# Autodesk Inventor assembly: Final2
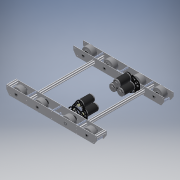
[picture p0: Inventor's stored thumbnail of the model, 180x180]
Saved by Autodesk Inventor 2016 (Build 200138000, 138)
## iProperties
Created: 2017-01-21
Part Number: Final2
Document SubType Name: Assembly
Designer: hamblettk
Author: hamblettk
## Documents named in this file (9)
- E:\1073CAD\Robot2017\DriveTrain\Final2.iam
- E:\1073CAD\Robot2017\DriveTrain\OutsidePlate2.ipt
- E:\1073CAD\Robot2017\DriveTrain\Individual Parts\3.625Churro.ipt
- E:\1073CAD\Robot2017\DriveTrain\Individual Parts\Mock 8020 3.375in.ipt
- E:\1073CAD\Robot2017\DriveTrain\InsidePlate2.ipt
- E:\1073CAD\Robot2017\DriveTrain\Individual Parts\Mock 8020 28.25in.ipt
- E:\1073CAD\Robot2017\DriveTrain\Individual Parts\DoublePulleyGearbox.iam
- E:\1073CAD\Robot2017\DriveTrain\Individual Parts\SinglePulley.iam
- E:\1073CAD\Robot2017\DriveTrain\Individual Parts\DoublePulley.iam
## Components (32 placed, 8 different names)
1. OutsidePlate2:1 — Mate:1, Mate:2, Mate:3, Mate:4, Mate:5, Mate:6, Mate:7, Mate:8, Mate:9, Mate:10, Flush:1, Flush:2, Mate:12, Mate:13, Mate:29, Mate:30, Mate:32, Mate:33, Mate:36, Mate:37, Mate:40, Mate:41
2. 3.625Churro:1 — Mate:1
3. 3.625Churro:2 — Mate:8
4. 3.625Churro:3 — Mate:7
5. 3.625Churro:4 — Mate:6
6. 3.625Churro:5 — Mate:4
7. 3.625Churro:6 — Mate:5
8. 3.625Churro:7 — Mate:2
9. 3.625Churro:8 — Mate:3
10. Mock 8020 3.375in:1 — Mate:9, Mate:11
11. Mock 8020 3.375in:2 — Mate:10
12. InsidePlate2:1 — Mate:11, Flush:1, Flush:2, Mate:31
13. Mock 8020 28.25in:1 — Mate:13, Mate:15, Mate:16
14. Mock 8020 28.25in:2 — Mate:12, Mate:14
15. OutsidePlate2:2 — Mate:14, Mate:15, Mate:16, Flush:3, Flush:4, Mate:25, Mate:26, Mate:27, Mate:42, Mate:43
16. InsidePlate2:2 — Flush:3, Flush:4, Mate:17, Mate:18, Mate:19, Mate:20, Mate:21, Mate:22, Mate:23, Mate:24, Mate:28, Mate:34, Mate:35, Mate:38, Mate:39
17. 3.625Churro:9 — Mate:17
18. 3.625Churro:10 — Mate:18
19. 3.625Churro:11 — Mate:19
20. 3.625Churro:12 — Mate:20, Mate:25
21. 3.625Churro:13 — Mate:21
22. 3.625Churro:14 — Mate:22
23. 3.625Churro:15 — Mate:23
24. 3.625Churro:16 — Mate:24
25. DoublePulleyGearbox:1 [sub-assembly] — Mate:29, Mate:30, Mate:31
26. DoublePulleyGearbox:2 [sub-assembly] — Mate:26, Mate:27, Mate:28
27. SinglePulley:1 [sub-assembly] — Mate:32, Mate:33
28. SinglePulley:2 [sub-assembly] — Mate:36, Mate:37
29. SinglePulley:3 [sub-assembly] — Mate:38, Mate:39
30. SinglePulley:4 [sub-assembly] — Mate:34, Mate:35
31. DoublePulley:1 [sub-assembly] — Mate:40, Mate:41
32. DoublePulley:2 [sub-assembly] — Mate:42, Mate:43
## Relationships (47: Mate 43, Flush 4)
- Mate:1: OutsidePlate2:1 ↔ 3.625Churro:1
- Mate:2: OutsidePlate2:1 ↔ 3.625Churro:7
- Mate:3: OutsidePlate2:1 ↔ 3.625Churro:8
- Mate:4: OutsidePlate2:1 ↔ 3.625Churro:5
- Mate:5: OutsidePlate2:1 ↔ 3.625Churro:6
- Mate:6: OutsidePlate2:1 ↔ 3.625Churro:4
- Mate:7: OutsidePlate2:1 ↔ 3.625Churro:3
- Mate:8: OutsidePlate2:1 ↔ 3.625Churro:2
- Mate:9: OutsidePlate2:1 ↔ Mock 8020 3.375in:1
- Mate:10: OutsidePlate2:1 ↔ Mock 8020 3.375in:2
- Mate:11: Mock 8020 3.375in:1 ↔ InsidePlate2:1
- Flush:1: OutsidePlate2:1 ↔ InsidePlate2:1
- Flush:2: OutsidePlate2:1 ↔ InsidePlate2:1
- Mate:12: OutsidePlate2:1 ↔ Mock 8020 28.25in:2
- Mate:13: OutsidePlate2:1 ↔ Mock 8020 28.25in:1
- Mate:14: Mock 8020 28.25in:2 ↔ OutsidePlate2:2
- Mate:15: Mock 8020 28.25in:1 ↔ OutsidePlate2:2
- Mate:16: Mock 8020 28.25in:1 ↔ OutsidePlate2:2
- Flush:3: OutsidePlate2:2 ↔ InsidePlate2:2
- Flush:4: OutsidePlate2:2 ↔ InsidePlate2:2
- Mate:17: InsidePlate2:2 ↔ 3.625Churro:9
- Mate:18: InsidePlate2:2 ↔ 3.625Churro:10
- Mate:19: InsidePlate2:2 ↔ 3.625Churro:11
- Mate:20: InsidePlate2:2 ↔ 3.625Churro:12
- Mate:21: InsidePlate2:2 ↔ 3.625Churro:13
- Mate:22: InsidePlate2:2 ↔ 3.625Churro:14
- Mate:23: InsidePlate2:2 ↔ 3.625Churro:15
- Mate:24: InsidePlate2:2 ↔ 3.625Churro:16
- Mate:25: OutsidePlate2:2 ↔ 3.625Churro:12
- Mate:26: OutsidePlate2:2 ↔ DoublePulleyGearbox:2
- Mate:27: OutsidePlate2:2 ↔ DoublePulleyGearbox:2
- Mate:28: InsidePlate2:2 ↔ DoublePulleyGearbox:2
- Mate:29: OutsidePlate2:1 ↔ DoublePulleyGearbox:1
- Mate:30: OutsidePlate2:1 ↔ DoublePulleyGearbox:1
- Mate:31: InsidePlate2:1 ↔ DoublePulleyGearbox:1
- Mate:32: OutsidePlate2:1 ↔ SinglePulley:1
- Mate:33: OutsidePlate2:1 ↔ SinglePulley:1
- Mate:34: InsidePlate2:2 ↔ SinglePulley:4
- Mate:35: InsidePlate2:2 ↔ SinglePulley:4
- Mate:36: OutsidePlate2:1 ↔ SinglePulley:2
- Mate:37: OutsidePlate2:1 ↔ SinglePulley:2
- Mate:38: InsidePlate2:2 ↔ SinglePulley:3
- Mate:39: InsidePlate2:2 ↔ SinglePulley:3
- Mate:40: OutsidePlate2:1 ↔ DoublePulley:1
- Mate:41: OutsidePlate2:1 ↔ DoublePulley:1
- Mate:42: OutsidePlate2:2 ↔ DoublePulley:2
- Mate:43: OutsidePlate2:2 ↔ DoublePulley:2
